# Autodesk Inventor assembly: 775pro_0_Female
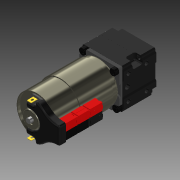
[picture p0: Inventor's stored thumbnail of the model, 180x180]
Saved by Autodesk Inventor 2022 (Build 260153000, 153)
## iProperties
Created: 2018-08-19
Part Number: 775pro_0_Female
Document SubType Name: Assembly
Mass: 1123.04 g
Surface Area: 1203.25 cm^2
Volume: 285.054 cm^3
Density: 3.93975 g/cm^3
## Documents named in this file (9)
- C:\Users\Cal\Desktop\Robotics\Design\Collaborative\Collaborative Parts Library\General Gearboxes\Planetaries\Versaplanetary\VersaPlanetary\775pro, 0 Stages, Female Output.iam
- C:\Users\Cal\Desktop\Robotics\Design\Collaborative\Collaborative Parts Library\General Gearboxes\Planetaries\Versaplanetary\V2 Stages\V2 Output Stage.iam
- C:\Users\Cal\Desktop\Robotics\Design\Collaborative\Collaborative Parts Library\General Gearboxes\Planetaries\Versaplanetary\V2 Stages\V2 Input Stage.iam
- C:\Users\Cal\Desktop\Robotics\Design\Collaborative\Collaborative Parts Library\General Gearboxes\Planetaries\Versaplanetary\Screws\8-32 x 1.25in Screw.ipt
- C:\Users\Cal\Desktop\Robotics\Design\Collaborative\Collaborative Parts Library\Power Transfer\Bearings and Bushings\Bearings\6902ZZ.ipt
- E:\Middleton Robotics\Collaborative Robots\Collaborative Part Library\Power Transfer\Bearings.ipt
- C:\Users\Cal\Desktop\Robotics\Design\Collaborative\Collaborative Parts Library\General Gearboxes\Planetaries\Versaplanetary\V2 Stages\V2 Input Stage\VP 775pro Input.iam
- C:\Users\Cal\Desktop\Robotics\Design\Collaborative\Collaborative Parts Library\General Gearboxes\Planetaries\Versaplanetary\VersaPlanetary.iam
- C:\Users\Cal\Desktop\Robotics\Design\Collaborative\Collaborative Parts Library\General Gearboxes\Planetaries\Versaplanetary\V2 Stages\V2 Output Stage\VP V2 Output Stage Female.iam
## Components (6 placed, 4 different names)
1. VP V2 Output Stage Female:3 [sub-assembly] — 0StageBasicInputMate1, 0StageBasicInputMate2, 0StageBasicInputMate3, Insert:25
2. VP 775pro Input:1 [sub-assembly] — 0StageBasicInputMate1, 0StageBasicInputMate2, 0StageBasicInputMate3, Insert:12, Insert:13
3. 8-32 x 1.25in Screw:1 — Insert:12
4. 8-32 x 1.25in Screw:2 — Insert:13
5. 6902ZZ:1
6. 6902ZZ:2 — Insert:25
## Relationships (6: Insert 3, Flush 2, Mate 1)
- 0StageBasicInputMate1 [Mate]: VP V2 Output Stage Female:3 ↔ VP 775pro Input:1
- 0StageBasicInputMate2 [Flush]: VP V2 Output Stage Female:3 ↔ VP 775pro Input:1
- 0StageBasicInputMate3 [Flush]: VP V2 Output Stage Female:3 ↔ VP 775pro Input:1
- Insert:12: VP 775pro Input:1 ↔ 8-32 x 1.25in Screw:1
- Insert:13: VP 775pro Input:1 ↔ 8-32 x 1.25in Screw:2
- Insert:25: VP V2 Output Stage Female:3 ↔ 6902ZZ:2
